# Autodesk Inventor assembly: StorageAssembly.ver4-1111-2020
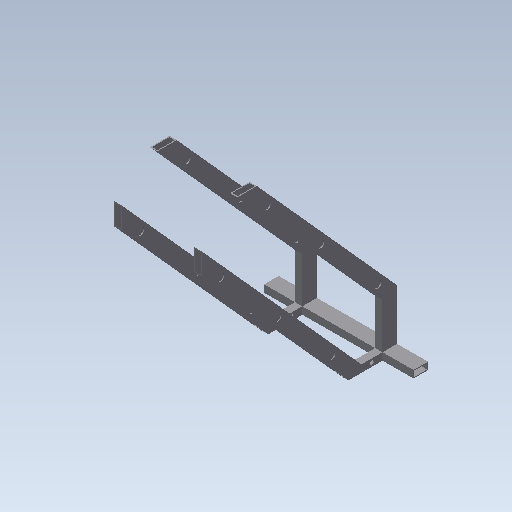
[picture p0: Inventor's stored thumbnail of the model, 512x512]
Saved by Autodesk Inventor 2021 (Build 250183000, 183)
## iProperties
Created: 2020-01-21
Part Number: StorageAssembly.ver4-1111-2020
Document SubType Name: Assembly
Designer: Power Hawks CADD
Author: Power Hawks CADD
## Documents named in this file (6)
- E:\PHRC CADD 2021\PHRC CADD\2020 Infinite Recharge\Storage\Assemblies\StorageAssembly.ver4-1111-2020.iam
- E:\PHRC CADD 2021\PHRC CADD\2020 Infinite Recharge\Shooting\Parts\SmallAnglesSupport.ver1-1111-2020.ipt
- E:\PHRC CADD 2021\PHRC CADD\2020 Infinite Recharge\Shooting\Parts\AngleBrace.ver1-1111-2020_MIR.ipt
- E:\PHRC CADD 2021\PHRC CADD\2020 Infinite Recharge\Shooting\Parts\SmallAnglesSupport.ver1-1111-2020_MIR.ipt
- E:\PHRC CADD 2021\PHRC CADD\2020 Infinite Recharge\Storage\Assemblies\StorageAssembly.ver3-1111-2020.iam
- E:\PHRC CADD 2021\PHRC CADD\2020 Infinite Recharge\Storage\Parts\IntakeBrace.ver1-1111-2020.ipt
## Components (6 placed, 5 different names)
1. SmallAnglesSupport.ver1-1111-2020:1 — Mate:6, Flush:8, Flush:9, Mate:10, Flush:10, Mate:11, Flush:11, Flush:12
2. AngleBrace.ver1-1111-2020_MIR:1
3. SmallAnglesSupport.ver1-1111-2020_MIR:1 — Mate:4, Flush:9
4. StorageAssembly.ver3-1111-2020:1 [sub-assembly] — Mate:4, Mate:6, Mate:8, Flush:7, Flush:10
5. IntakeBrace.ver1-1111-2020:1 — Mate:8, Flush:7, Flush:8, Mate:10
6. AngleBrace.ver1-1111-2020_MIR:2 — Mate:11, Flush:11, Flush:12
## Relationships (13: Flush 8, Mate 5)
- [Flush]: AngleBrace.ver1-1111-2020_MIR:1 ↔ SmallAnglesSupport.ver1-1111-2020_MIR:1
- [Flush]: AngleBrace.ver1-1111-2020_MIR:1 ↔ SmallAnglesSupport.ver1-1111-2020_MIR:1
- Mate:4: SmallAnglesSupport.ver1-1111-2020_MIR:1 ↔ StorageAssembly.ver3-1111-2020:1
- Mate:6: SmallAnglesSupport.ver1-1111-2020:1 ↔ StorageAssembly.ver3-1111-2020:1
- Mate:8: StorageAssembly.ver3-1111-2020:1 ↔ IntakeBrace.ver1-1111-2020:1
- Flush:7: StorageAssembly.ver3-1111-2020:1 ↔ IntakeBrace.ver1-1111-2020:1
- Flush:8 (107.95 mm): SmallAnglesSupport.ver1-1111-2020:1 ↔ IntakeBrace.ver1-1111-2020:1
- Flush:9: SmallAnglesSupport.ver1-1111-2020:1 ↔ SmallAnglesSupport.ver1-1111-2020_MIR:1
- Mate:10: SmallAnglesSupport.ver1-1111-2020:1 ↔ IntakeBrace.ver1-1111-2020:1
- Flush:10: SmallAnglesSupport.ver1-1111-2020:1 ↔ StorageAssembly.ver3-1111-2020:1
- Mate:11: SmallAnglesSupport.ver1-1111-2020:1 ↔ AngleBrace.ver1-1111-2020_MIR:2
- Flush:11: SmallAnglesSupport.ver1-1111-2020:1 ↔ AngleBrace.ver1-1111-2020_MIR:2
- Flush:12: SmallAnglesSupport.ver1-1111-2020:1 ↔ AngleBrace.ver1-1111-2020_MIR:2
